# Autodesk Inventor assembly: EDM Machine+Shields
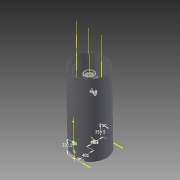
[picture p0: Inventor's stored thumbnail of the model, 180x180]
Saved by Autodesk Inventor 2015 (Build 190159000, 159)
## iProperties
Created: 2014-10-03
Part Number: EDM Machine+Shields
Document SubType Name: Assembly
Designer: I Rabey
Author: I Rabey
## Documents named in this file (12)
- C:\ColdMatter\CADFiles\EDM Machine\EDM Machine+Shields.iam
- C:\ColdMatter\CADFiles\EDM Machine\EDM Beamline\Chamber parts\hudson chamber actual size.ipt
- C:\ColdMatter\CADFiles\EDM Machine\EDM Beamline\Chamber parts\Centre nipple.iam
- C:\ColdMatter\CADFiles\EDM Machine\Electrical Feedthrough Collar\Electrical Feedthrough Collar.iam
- C:\ColdMatter\CADFiles\EDM Machine\Microwave Detection Region\Detection Region Chamber.iam
- C:\ColdMatter\CADFiles\EDM Machine\EDM Inner Shield\Inner Shield.iam
- C:\ColdMatter\CADFiles\EDM Machine\Microwave Detection Region\Probe Shield\Probe Shield Design.iam
- C:\ColdMatter\CADFiles\EDM Machine\EDM Middle Shield\Lower Front Half 2014 Replacement.ipt
- C:\ColdMatter\CADFiles\EDM Machine\EDM Middle Shield\Lower Back Half 2014 Replacement.ipt
- C:\ColdMatter\CADFiles\EDM Machine\EDM Middle Shield\Upper Front Half 2014 Replacement.ipt
- C:\ColdMatter\CADFiles\EDM Machine\EDM Middle Shield\Upper Back Half 2014 Replacement.ipt
- C:\ColdMatter\CADFiles\EDM Machine\EDM Outer Shield\Outer Shield.iam
## Components (11 placed, 11 different names)
1. hudson chamber actual size:1 — Mate:13, Mate:14, Mate:15, Mate:16, Mate:35, Mate:36
2. Centre nipple:1 [sub-assembly] — Mate:5, Mate:6, Mate:13, Mate:14
3. Electrical Feedthrough Collar:1 [sub-assembly] — Mate:5, Mate:6, Mate:7, Mate:8, Mate:9, Mate:34
4. Detection Region Chamber:1 [sub-assembly] — Mate:8, Mate:9, Mate:10, Mate:11, Mate:17, Mate:18
5. Inner Shield:1 [sub-assembly] — Mate:11, Mate:12, Mate:16
6. Probe Shield Design:1 [sub-assembly] — Mate:17, Mate:18
7. Lower Front Half 2014 Replacement:1 — Mate:38, Mate:39
8. Lower Back Half 2014 Replacement:1 — Mate:35, Mate:36, Mate:37, Mate:38, Mate:42
9. Upper Front Half 2014 Replacement:1 — Mate:34, Mate:37, Mate:40, Mate:41
10. Upper Back Half 2014 Replacement:1 — Mate:39, Mate:40, Mate:41, Mate:43
11. Outer Shield:1 [sub-assembly] — Mate:42, Mate:43
## Relationships (24: Mate 24)
- Mate:5: Centre nipple:1 ↔ Electrical Feedthrough Collar:1
- Mate:6: Centre nipple:1 ↔ Electrical Feedthrough Collar:1
- Mate:7: Electrical Feedthrough Collar:1
- Mate:8: Electrical Feedthrough Collar:1 ↔ Detection Region Chamber:1
- Mate:9: Electrical Feedthrough Collar:1 ↔ Detection Region Chamber:1
- Mate:10: Detection Region Chamber:1
- Mate:11: Detection Region Chamber:1 ↔ Inner Shield:1
- Mate:12: Inner Shield:1
- Mate:13: hudson chamber actual size:1 ↔ Centre nipple:1
- Mate:14: hudson chamber actual size:1 ↔ Centre nipple:1
- Mate:15: hudson chamber actual size:1
- Mate:16: hudson chamber actual size:1 ↔ Inner Shield:1
- Mate:17: Detection Region Chamber:1 ↔ Probe Shield Design:1
- Mate:18: Detection Region Chamber:1 ↔ Probe Shield Design:1
- Mate:34: Electrical Feedthrough Collar:1 ↔ Upper Front Half 2014 Replacement:1
- Mate:35: hudson chamber actual size:1 ↔ Lower Back Half 2014 Replacement:1
- Mate:36: hudson chamber actual size:1 ↔ Lower Back Half 2014 Replacement:1
- Mate:37: Lower Back Half 2014 Replacement:1 ↔ Upper Front Half 2014 Replacement:1
- Mate:38: Lower Front Half 2014 Replacement:1 ↔ Lower Back Half 2014 Replacement:1
- Mate:39: Lower Front Half 2014 Replacement:1 ↔ Upper Back Half 2014 Replacement:1
- Mate:40: Upper Front Half 2014 Replacement:1 ↔ Upper Back Half 2014 Replacement:1
- Mate:41: Upper Front Half 2014 Replacement:1 ↔ Upper Back Half 2014 Replacement:1
- Mate:42: Lower Back Half 2014 Replacement:1 ↔ Outer Shield:1
- Mate:43: Upper Back Half 2014 Replacement:1 ↔ Outer Shield:1
